# Autodesk Inventor assembly: main
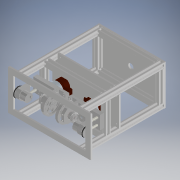
[picture p0: Inventor's stored thumbnail of the model, 180x180]
Saved by Autodesk Inventor 2020 (Build 240168000, 168)
## iProperties
Created: 2019-11-21
Part Number: main
Document SubType Name: Assembly
Designer: bapti
Author: bapti
## Documents named in this file (8)
- C:\Users\bapti\Documents\Inventor\EIRBOT_sailtheworld\robot\main.iam
- C:\Users\bapti\Documents\Inventor\EIRBOT_sailtheworld\robot\floor.ipt
- C:\Users\bapti\Documents\Inventor\EIRBOT_sailtheworld\robot\top.ipt
- C:\Users\bapti\Documents\Inventor\EIRBOT_sailtheworld\robot\AP20x20_Z.ipt
- C:\Users\bapti\Documents\Inventor\EIRBOT_sailtheworld\robot\AP20x20_X.ipt
- C:\Users\bapti\Documents\Inventor\EIRBOT_sailtheworld\robot\AP20x20_Y.ipt
- C:\Users\bapti\Documents\Inventor\EIRBOT_sailtheworld\robot\patin.ipt
- C:\Users\bapti\Documents\Inventor\EIRBOT_sailtheworld\moteur\moteurEncodeurRoues.ipt
## Components (17 placed, 7 different names)
1. floor:1 — Placage:8, Placage:9
2. top:1 — Placage:4, Affleurement:1, Affleurement:2, Placage:5, Placage:6, Placage:7, Affleurement:3, Affleurement:4, Affleurement:5, Affleurement:6, Affleurement:7, Affleurement:8, Placage:18, Placage:19, Placage:20, Placage:21
3. AP20x20_Z:1 — Placage:1, Placage:2, Placage:3, Placage:4, Affleurement:1, Affleurement:2, Placage:8, Placage:9, Placage:16, Affleurement:15, Affleurement:16, Placage:17, Placage:22, Affleurement:20, Affleurement:21, Placage:25
4. AP20x20_Z:2 — Placage:7, Affleurement:3, Affleurement:4
5. AP20x20_Z:3 — Placage:6, Affleurement:7, Affleurement:8, Placage:10, Placage:11, Affleurement:11, Affleurement:12, Placage:14, Affleurement:13, Affleurement:14, Placage:15, Placage:24
6. AP20x20_Z:4 — Placage:5, Affleurement:5, Affleurement:6, Placage:12, Placage:13, Affleurement:9, Affleurement:10
7. AP20x20_X:1 — Placage:12, Affleurement:10, Placage:19
8. AP20x20_X:2 — Placage:13, Affleurement:9, Affleurement:18, Affleurement:19
9. AP20x20_X:3 — Placage:14, Affleurement:13, Placage:20
10. AP20x20_X:4 — Affleurement:14, Placage:15, Affleurement:18
11. AP20x20_Y:1 — Placage:16, Affleurement:15, Placage:18
12. AP20x20_Y:2 — Affleurement:16, Placage:17, Affleurement:17, Affleurement:19, Placage:23
13. AP20x20_Y:3 — Placage:10, Affleurement:11, Placage:21
14. AP20x20_Y:4 — Placage:11, Affleurement:12, Affleurement:17
15. patin:1 — Placage:22, Affleurement:20, Affleurement:21, Tangente:1
16. moteurEncodeurRoues:1 — Affleurement:22, Affleurement:23, Placage:23, Placage:25
17. moteurEncodeurRoues:2 — Affleurement:22, Affleurement:23, Tangente:1, Placage:24
## Relationships (49: Mate 25, Flush 23, Tangent 1)
- Placage:1 [Mate]: AP20x20_Z:1
- Placage:2 [Mate]: AP20x20_Z:1
- Placage:3 [Mate]: AP20x20_Z:1
- Placage:4 [Mate]: top:1 ↔ AP20x20_Z:1
- Affleurement:1 [Flush]: top:1 ↔ AP20x20_Z:1
- Affleurement:2 [Flush]: top:1 ↔ AP20x20_Z:1
- Placage:5 [Mate]: top:1 ↔ AP20x20_Z:4
- Placage:6 [Mate]: top:1 ↔ AP20x20_Z:3
- Placage:7 [Mate]: top:1 ↔ AP20x20_Z:2
- Affleurement:3 [Flush]: top:1 ↔ AP20x20_Z:2
- Affleurement:4 [Flush]: top:1 ↔ AP20x20_Z:2
- Affleurement:5 [Flush]: top:1 ↔ AP20x20_Z:4
- Affleurement:6 [Flush]: top:1 ↔ AP20x20_Z:4
- Affleurement:7 [Flush]: top:1 ↔ AP20x20_Z:3
- Affleurement:8 [Flush]: top:1 ↔ AP20x20_Z:3
- Placage:8 [Mate]: floor:1 ↔ AP20x20_Z:1
- Placage:9 [Mate]: floor:1 ↔ AP20x20_Z:1
- Placage:10 [Mate]: AP20x20_Z:3 ↔ AP20x20_Y:3
- Placage:11 [Mate]: AP20x20_Z:3 ↔ AP20x20_Y:4
- Placage:12 [Mate]: AP20x20_Z:4 ↔ AP20x20_X:1
- Placage:13 [Mate]: AP20x20_Z:4 ↔ AP20x20_X:2
- Affleurement:9 [Flush]: AP20x20_Z:4 ↔ AP20x20_X:2
- Affleurement:10 [Flush]: AP20x20_Z:4 ↔ AP20x20_X:1
- Affleurement:11 [Flush]: AP20x20_Z:3 ↔ AP20x20_Y:3
- Affleurement:12 [Flush]: AP20x20_Z:3 ↔ AP20x20_Y:4
- Placage:14 [Mate]: AP20x20_Z:3 ↔ AP20x20_X:3
- Affleurement:13 [Flush]: AP20x20_Z:3 ↔ AP20x20_X:3
- Affleurement:14 [Flush]: AP20x20_Z:3 ↔ AP20x20_X:4
- Placage:15 [Mate]: AP20x20_Z:3 ↔ AP20x20_X:4
- Placage:16 [Mate]: AP20x20_Z:1 ↔ AP20x20_Y:1
- Affleurement:15 [Flush]: AP20x20_Z:1 ↔ AP20x20_Y:1
- Affleurement:16 [Flush]: AP20x20_Z:1 ↔ AP20x20_Y:2
- Placage:17 [Mate]: AP20x20_Z:1 ↔ AP20x20_Y:2
- Placage:18 [Mate]: top:1 ↔ AP20x20_Y:1
- Placage:19 [Mate]: top:1 ↔ AP20x20_X:1
- Placage:20 [Mate]: top:1 ↔ AP20x20_X:3
- Placage:21 [Mate]: top:1 ↔ AP20x20_Y:3
- Affleurement:17 [Flush]: AP20x20_Y:2 ↔ AP20x20_Y:4
- Affleurement:18 [Flush]: AP20x20_X:2 ↔ AP20x20_X:4
- Affleurement:19 [Flush]: AP20x20_X:2 ↔ AP20x20_Y:2
- Placage:22 [Mate]: AP20x20_Z:1 ↔ patin:1
- Affleurement:20 [Flush]: AP20x20_Z:1 ↔ patin:1
- Affleurement:21 [Flush] (-30 mm): AP20x20_Z:1 ↔ patin:1
- Affleurement:22 [Flush]: moteurEncodeurRoues:1 ↔ moteurEncodeurRoues:2
- Affleurement:23 [Flush]: moteurEncodeurRoues:1 ↔ moteurEncodeurRoues:2
- Placage:23 [Mate] (25 mm): AP20x20_Y:2 ↔ moteurEncodeurRoues:1
- Tangente:1: patin:1 ↔ moteurEncodeurRoues:2
- Placage:24 [Mate]: AP20x20_Z:3 ↔ moteurEncodeurRoues:2
- Placage:25 [Mate]: AP20x20_Z:1 ↔ moteurEncodeurRoues:1
